# Autodesk Inventor assembly: ensambleDedo
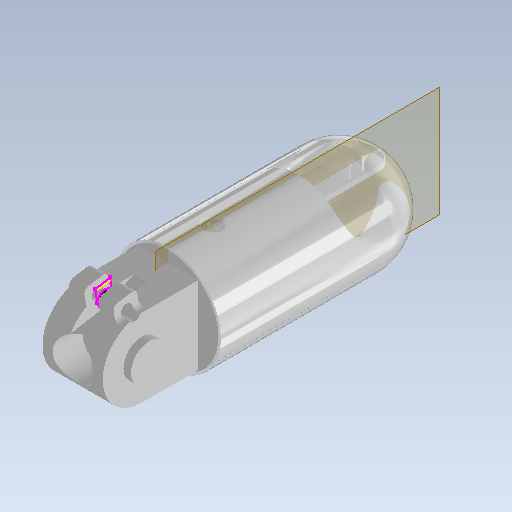
[picture p0: Inventor's stored thumbnail of the model, 512x512]
Saved by Autodesk Inventor 2021 (Build 250183000, 183)
## iProperties
Created: 2023-08-28
Part Number: ensambleDedo
Document SubType Name: Assembly
Designer: Sergio
Author: Sergio
## Documents named in this file (7)
- D:\Sergio\OneDrive - Escuela Superior Politécnica del Litoral\Documentos\12vo Semestre (último)\Diseño Mecatrónico\Proyecto\Diseño Mecánico\solucion GANADORA\dedo\Dedo.iam
- D:\Sergio\OneDrive - Escuela Superior Politécnica del Litoral\Documentos\12vo Semestre (último)\Diseño Mecatrónico\Proyecto\Diseño Mecánico\solucion GANADORA\dedo\celda de carga.ipt
- D:\Sergio\OneDrive - Escuela Superior Politécnica del Litoral\Documentos\12vo Semestre (último)\Diseño Mecatrónico\Proyecto\Diseño Mecánico\solucion GANADORA\dedo\Junta de dedo.ipt
- D:\Sergio\OneDrive - Escuela Superior Politécnica del Litoral\Documentos\12vo Semestre (último)\Diseño Mecatrónico\Proyecto\Diseño Mecánico\solucion GANADORA\dedo\Dedo sección superior.ipt
- D:\Sergio\OneDrive - Escuela Superior Politécnica del Litoral\Documentos\12vo Semestre (último)\Diseño Mecatrónico\Proyecto\Diseño Mecánico\solucion GANADORA\dedo\Capa flexible.ipt
- D:\Sergio\Documents\Inventor\Content Center Files\R2021\es-ES\AS 1427(04)\AS 1427 - M2 x 8(5) I.ipt
- D:\Sergio\Documents\Inventor\Content Center Files\R2021\es-ES\AS 1427(04)\AS 1427 - M4 x 16(5) I.ipt
## Components (6 placed, 6 different names)
1. celda de carga:1 — Coincidencia:4, Coincidencia:5, Coincidencia:6
2. Junta de dedo:1 — Coincidencia:1, Coincidencia:7, Coincidencia:8
3. Dedo sección superior:1 — Insertar:1, Coincidencia:3, Coincidencia:4, Coincidencia:5, Coincidencia:7, Coincidencia:8, Insertar:2, Nivelación:10, Nivelación:11
4. Capa flexible:1 — Insertar:2, Nivelación:10
5. AS 1427 H - Métrico M4 x 16:1 — Coincidencia:1, Insertar:1
6. AS 1427 H - Métrico M2 x 8:1 — Coincidencia:3, Coincidencia:6
## Relationships (11: Mate 7, Insert 2, Flush 2)
- Coincidencia:1 [Mate]: Junta de dedo:1 ↔ AS 1427 H - Métrico M4 x 16:1
- Insertar:1: Dedo sección superior:1 ↔ AS 1427 H - Métrico M4 x 16:1
- Coincidencia:3 [Mate]: Dedo sección superior:1 ↔ AS 1427 H - Métrico M2 x 8:1
- Coincidencia:4 [Mate]: celda de carga:1 ↔ Dedo sección superior:1
- Coincidencia:5 [Mate]: celda de carga:1 ↔ Dedo sección superior:1
- Coincidencia:6 [Mate]: celda de carga:1 ↔ AS 1427 H - Métrico M2 x 8:1
- Coincidencia:7 [Mate]: Junta de dedo:1 ↔ Dedo sección superior:1
- Coincidencia:8 [Mate]: Junta de dedo:1 ↔ Dedo sección superior:1
- Insertar:2: Dedo sección superior:1 ↔ Capa flexible:1
- Nivelación:10 [Flush]: Dedo sección superior:1 ↔ Capa flexible:1
- Nivelación:11 [Flush]: Dedo sección superior:1
